# Autodesk Inventor assembly: Weapon (Motor-Side Pulley)
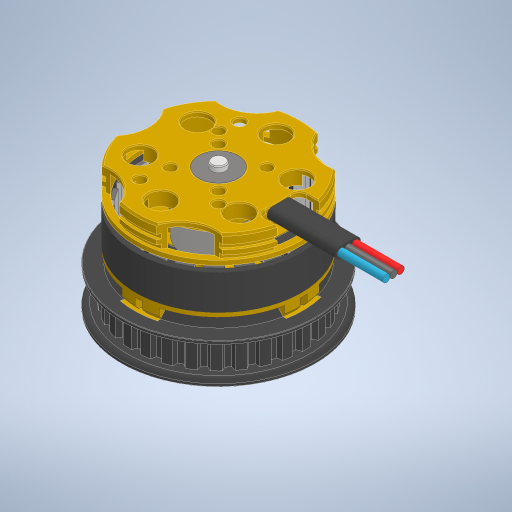
[picture p0: Inventor's stored thumbnail of the model, 512x512]
Saved by Autodesk Inventor 2023.2 (Build 272271000, 271)
## iProperties
Created: 2022-05-21
Part Number: Weapon (Motor-Side Pulley)
Document SubType Name: Assembly
Designer: Nathan Cai
Mass: 47.0942 g
Surface Area: 258.644 cm^2
Volume: 28.2879 cm^3
Density: 1.66481 g/cm^3
Author: Nathan Cai
## Documents named in this file (3)
- C:\Users\Nathan Cai\Documents\Inventor\0.3rd Lawette - V3.6\Vertical Weapon Assembly (Type A - Low Power)\Weapon (Motor-Side Pulley).iam
- C:\Users\Nathan Cai\Documents\Inventor\0.3rd Lawette - V3.6\Vertical Weapon Assembly (Type A - Low Power)\XL Pulley 30T .25in Wd.ipt
- C:\Users\Nathan Cai\Documents\Inventor\0.3rd Lawette - V3.6\FEICHAO BE4108 380KV\FEICHAO BE4108 380KV.iam
## Components (2 placed, 2 different names)
1. XL Pulley 30T .25in Wd:1 — Mate:2, Mate:3, Mate:4
2. FEICHAO BE4108 380KV:1 [sub-assembly] — Mate:2, Mate:3, Mate:4
## Relationships (3: Mate 3)
- Mate:2 (-33.9996 mm): XL Pulley 30T .25in Wd:1 ↔ FEICHAO BE4108 380KV:1
- Mate:3: XL Pulley 30T .25in Wd:1 ↔ FEICHAO BE4108 380KV:1
- Mate:4: XL Pulley 30T .25in Wd:1 ↔ FEICHAO BE4108 380KV:1
